# Autodesk Inventor assembly: Pipe Assy
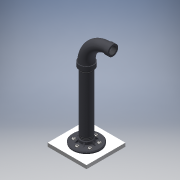
[picture p0: Inventor's stored thumbnail of the model, 180x180]
Saved by Autodesk Inventor 2019 (Build 230136000, 136)
## iProperties
Created: 2019-08-29
Part Number: Pipe Assy
Document SubType Name: Assembly
Designer: Rick Szalay
Author: Rick Szalay
## Documents named in this file (6)
- C:\Users\Rick Szalay\Documents\Inventor\CAD Basix\Pipe Assy.iam
- C:\Users\Rick Szalay\Documents\Inventor\CAD Basix\2 Inch Pipe Flange.ipt
- C:\Users\Rick Szalay\Documents\Inventor\CAD Basix\2 Inch Pipe.ipt
- C:\Users\Rick Szalay\Documents\Inventor\CAD Basix\2-1.25 Inch Elbow Adapter.ipt
- C:\Users\Rick Szalay\Documents\Inventor\CAD Basix\Mounting Plate.ipt
- C:\Users\Rick Szalay\Documents\Inventor\Content Center Files\R2019\en-US\ANSI B18.3(03)\ANSI B18.3 - 3_8-24 UNF - UNF - 0.875(1).ipt
## Components (10 placed, 5 different names)
1. 2 Inch Pipe Flange:1 — Mate:1, Mate:2, Mate:3, Mate:6, Insert:1, Insert:2, Insert:3, Insert:4, Insert:5, Insert:6
2. 2 Inch Pipe:1 — Mate:2, Mate:3, Mate:4, Mate:5, Mate:7
3. 2-1.25 Inch Elbow Adapter:1 — Mate:4, Mate:5, Angle:1
4. Mounting Plate:1 — Mate:6, Mate:7, Angle:2
5. Hexagon Socket Button Head Cap Screw - Inch 3/8-24 - 7/8:1 — Insert:1
6. Hexagon Socket Button Head Cap Screw - Inch 3/8-24 - 7/8:2 — Insert:2
7. Hexagon Socket Button Head Cap Screw - Inch 3/8-24 - 7/8:3 — Insert:3
8. Hexagon Socket Button Head Cap Screw - Inch 3/8-24 - 7/8:4 — Insert:4
9. Hexagon Socket Button Head Cap Screw - Inch 3/8-24 - 7/8:5 — Insert:5
10. Hexagon Socket Button Head Cap Screw - Inch 3/8-24 - 7/8:6 — Insert:6
## Relationships (15: Mate 7, Insert 6, Angle 2)
- Mate:1: 2 Inch Pipe Flange:1
- Mate:2: 2 Inch Pipe Flange:1 ↔ 2 Inch Pipe:1
- Mate:3 (-12.7 mm): 2 Inch Pipe Flange:1 ↔ 2 Inch Pipe:1
- Mate:4: 2 Inch Pipe:1 ↔ 2-1.25 Inch Elbow Adapter:1
- Mate:5 (-12.7 mm): 2 Inch Pipe:1 ↔ 2-1.25 Inch Elbow Adapter:1
- Angle:1 (0 deg): 2-1.25 Inch Elbow Adapter:1
- Mate:6: 2 Inch Pipe Flange:1 ↔ Mounting Plate:1
- Mate:7: 2 Inch Pipe:1 ↔ Mounting Plate:1
- Angle:2 (0 deg): Mounting Plate:1
- Insert:1: 2 Inch Pipe Flange:1 ↔ Hexagon Socket Button Head Cap Screw - Inch 3/8-24 - 7/8:1
- Insert:2: 2 Inch Pipe Flange:1 ↔ Hexagon Socket Button Head Cap Screw - Inch 3/8-24 - 7/8:2
- Insert:3: 2 Inch Pipe Flange:1 ↔ Hexagon Socket Button Head Cap Screw - Inch 3/8-24 - 7/8:3
- Insert:4: 2 Inch Pipe Flange:1 ↔ Hexagon Socket Button Head Cap Screw - Inch 3/8-24 - 7/8:4
- Insert:5: 2 Inch Pipe Flange:1 ↔ Hexagon Socket Button Head Cap Screw - Inch 3/8-24 - 7/8:5
- Insert:6: 2 Inch Pipe Flange:1 ↔ Hexagon Socket Button Head Cap Screw - Inch 3/8-24 - 7/8:6
